# Autodesk Inventor assembly: SplitterBoard
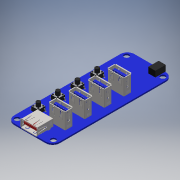
[picture p0: Inventor's stored thumbnail of the model, 180x180]
Saved by Autodesk Inventor 2019 (Build 230136000, 136)
## iProperties
Created: 2020-02-13
Part Number: SplitterBoard
Document SubType Name: Assembly
Designer: close
Author: close
## Documents named in this file (6)
- C:\Users\close\Desktop\CAD BARC-ROAR\barc_hardware\Dependencies\Splitter Board\SplitterBoard.iam
- C:\Users\close\Desktop\CAD BARC-ROAR\barc_hardware\Dependencies\Splitter Board\PCB.ipt
- C:\Users\close\Desktop\CAD BARC-ROAR\barc_hardware\Dependencies\Splitter Board\Tactal Switch - SMD (6mmx 6mmx 7mm) - Marked.ipt
- C:\Users\close\Desktop\CAD BARC-ROAR\barc_hardware\Dependencies\Splitter Board\USB type-A female 2.ipt
- C:\Users\close\Desktop\CAD BARC-ROAR\barc_hardware\Dependencies\Splitter Board\USB type-A female 1.ipt
- C:\Users\close\Desktop\CAD BARC-ROAR\barc_hardware\Dependencies\Splitter Board\Barrel Jack small.ipt
## Components (11 placed, 5 different names)
1. PCB:1 — Mate:1, Mate:2, Mate:3, Mate:4, Flush:4, Mate:8, Flush:5, Mate:9, Mate:10, Flush:10, Flush:11, Mate:17, Flush:12, Flush:13, Mate:18
2. Tactal Switch - SMD (6mmx 6mmx 7mm) - Marked:1 — Mate:1, Flush:1, Flush:4, Mate:5, Flush:13
3. Tactal Switch - SMD (6mmx 6mmx 7mm) - Marked:2 — Mate:4, Flush:1, Flush:2, Mate:5, Mate:6
4. Tactal Switch - SMD (6mmx 6mmx 7mm) - Marked:3 — Mate:3, Flush:2, Flush:3, Mate:6, Mate:7
5. Tactal Switch - SMD (6mmx 6mmx 7mm) - Marked:4 — Mate:2, Flush:3, Mate:7
6. USB type-A female 2:1 — Mate:8, Flush:5, Mate:9
7. Barrel Jack small:1 — Flush:11, Mate:17, Flush:12
8. USB type-A female 1:4 — Mate:10, Flush:10, Mate:18
9. USB type-A female 1:5
10. USB type-A female 1:6
11. USB type-A female 1:7
## Component patterns: (4 elements, first: USB type-A female 1:4)
## Relationships (21: Mate 12, Flush 9)
- Mate:1: PCB:1 ↔ Tactal Switch - SMD (6mmx 6mmx 7mm) - Marked:1
- Mate:2: PCB:1 ↔ Tactal Switch - SMD (6mmx 6mmx 7mm) - Marked:4
- Mate:3: PCB:1 ↔ Tactal Switch - SMD (6mmx 6mmx 7mm) - Marked:3
- Mate:4: PCB:1 ↔ Tactal Switch - SMD (6mmx 6mmx 7mm) - Marked:2
- Flush:1: Tactal Switch - SMD (6mmx 6mmx 7mm) - Marked:1 ↔ Tactal Switch - SMD (6mmx 6mmx 7mm) - Marked:2
- Flush:2: Tactal Switch - SMD (6mmx 6mmx 7mm) - Marked:2 ↔ Tactal Switch - SMD (6mmx 6mmx 7mm) - Marked:3
- Flush:3: Tactal Switch - SMD (6mmx 6mmx 7mm) - Marked:3 ↔ Tactal Switch - SMD (6mmx 6mmx 7mm) - Marked:4
- Flush:4 (17 mm): PCB:1 ↔ Tactal Switch - SMD (6mmx 6mmx 7mm) - Marked:1
- Mate:5 (11 mm): Tactal Switch - SMD (6mmx 6mmx 7mm) - Marked:1 ↔ Tactal Switch - SMD (6mmx 6mmx 7mm) - Marked:2
- Mate:6 (11 mm): Tactal Switch - SMD (6mmx 6mmx 7mm) - Marked:2 ↔ Tactal Switch - SMD (6mmx 6mmx 7mm) - Marked:3
- Mate:7 (11 mm): Tactal Switch - SMD (6mmx 6mmx 7mm) - Marked:3 ↔ Tactal Switch - SMD (6mmx 6mmx 7mm) - Marked:4
- Mate:8 (0.5 mm): PCB:1 ↔ USB type-A female 2:1
- Flush:5 (-13.3 mm): PCB:1 ↔ USB type-A female 2:1
- Mate:9 (-13.77 mm): PCB:1 ↔ USB type-A female 2:1
- Mate:10: PCB:1 ↔ USB type-A female 1:4
- Flush:10 (16.8 mm): PCB:1 ↔ USB type-A female 1:4
- Flush:11 (-0.5 mm): PCB:1 ↔ Barrel Jack small:1
- Mate:17: PCB:1 ↔ Barrel Jack small:1
- Flush:12 (6.7 mm): PCB:1 ↔ Barrel Jack small:1
- Flush:13 (4 mm): PCB:1 ↔ Tactal Switch - SMD (6mmx 6mmx 7mm) - Marked:1
- Mate:18 (6 mm): PCB:1 ↔ USB type-A female 1:4
